# Autodesk Inventor assembly: final_assembly_2017_SuperUltraLow
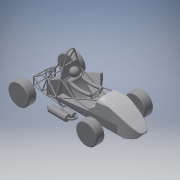
[picture p0: Inventor's stored thumbnail of the model, 180x180]
Saved by Autodesk Inventor 2018.1 (Build 221171000, 171)
## iProperties
Created: 2017-10-06
Part Number: final_assembly_2017_SuperUltraLow
Material: 一般
Document SubType Name: Assembly
Designer: kuwano
Sending System: Autodesk Inventor 2018
Preprocessor: ST-DEVELOPER v16.13
Title: D:\kuwano\Documents\Inventor\KITformula\CFD_KS-14\KS-14\stp\final_assembly_2017_SuperUltraLow.stp
Author: kuwano
## Documents named in this file (6)
- D:\formula\ドキュメント\Inventor\kuwano\KS-15\KS-14_SULow\KS-14_SULow.iam
- D:\formula\ドキュメント\Inventor\kuwano\KS-15\KS-14_SULow\parts\kaul_reretouch.ipt
- D:\formula\ドキュメント\Inventor\kuwano\KS-15\KS-14_SULow\parts\newbody.ipt
- D:\formula\ドキュメント\Inventor\kuwano\KS-15\KS-14_SULow\parts\tire_low.ipt
- D:\formula\ドキュメント\Inventor\kuwano\KS-15\KS-14_SULow\parts\tire_low_MIR.ipt
- D:\formula\ドキュメント\Inventor\kuwano\KS-15\KS-14_SULow\parts\driver.ipt
## Components (7 placed, 5 different names)
1. kaul_retouch:1 — メイト:1, メイト:2, メイト:3
2. newbody:1 — フラッシュ:4, メイト:1, メイト:2, メイト:3, メイト:4
3. tire_low:1
4. tire_low:2
5. tire_low_MIR:1
6. tire_low_MIR:2
7. driver:1 — メイト:4
## Relationships (5: Mate 4, Flush 1)
- フラッシュ:4 [Flush]: newbody:1
- メイト:1 [Mate]: kaul_retouch:1 ↔ newbody:1
- メイト:2 [Mate]: kaul_retouch:1 ↔ newbody:1
- メイト:3 [Mate]: kaul_retouch:1 ↔ newbody:1
- メイト:4 [Mate]: newbody:1 ↔ driver:1
